# Autodesk Inventor assembly: 2803622 EAMM-U-145-D100-120G-188-S1
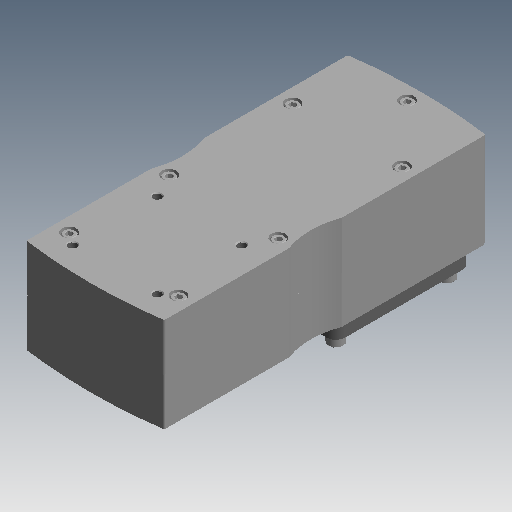
[picture p0: Inventor's stored thumbnail of the model, 512x512]
Saved by Autodesk Inventor 2021 (Build 250183000, 183)
## iProperties
Category: PARTsolutions
Company: FESTO
Part Number: 2803622 EAMM-U-145-D100-120G-188-S1
Catalog Web Link: www.cadenas.de
Description: EAMM-U-parallel kit
Vendor: FESTO
Document SubType Name: Assembly
Designer: partserver
Manufacturer: FESTO
Mass: 12100 g
Surface Area: 4483.28 cm^2
Volume: 3170.64 cm^3
Density: 3.81626 g/cm^3
PSOL_IDENT_0: {ATYP=ASSISTANT},{DATA=script=$CADENAS_DATA/23d-libs/festo/webfesto.vbb&M_FAMILY=EAMM&M_GROUP=01&M_P
PSOL_IDENT_1: ARTNO=2803622&IDCODE1=EAMM-U-145-D100-120G-188-S1&IDCODE2=&customer_number_cns=&MATES=1&LOD=HI&LOCKE
PSOL_IDENT_2: RP=0&SINGLEPART=1}
NB: 2803622 EAMM-U-145-D100-120G-188-S1
NN: EAMM-U
NT: parallel kit
NBSYN: $TNR. $TYP.
LINA: 2803622 EAMM-U-145-D100-120G-188-S1
CATALOG: Festo
TNR: 2803622
TYP: EAMM-U-145-D100-120G-188-S1
B1: 145
B2: 0
B3: 89
B4: 0
B5: 89
B6: 115
D1: 80
D2: 100
D3: 100
D4: 11
D5: 11
D6: M10
D7: 0
H1: 348
H2: 0
H3: 89
H4: 0
H5: 89
H6: 70
H7: 188
H8: 35
H9: 70
H10: 193
H11: 130
H12: 5
L1: 99.5
L2: 0.5
L3: 0
L4: 0
T1: 25
W1: 45
W2: 0
CNSMASSEXACT: 12.1
SUPPLIER: FESTO
ARTICLENO: 2803622 EAMM-U-145-D100-120G-188-S1
BOMINFO: 2803622 EAMM-U-145-D100-120G-188-S1
CREATOR: CADENAS GmbH
Title: 2803622 EAMM-U-145-D100-120G-188-S1
Author: Cadenas PARTsolutions
Comments: parallel kit
## Documents named in this file (11)
- C:\Users\Santiago Suárez\Documents\GitHub\Dis.-Mecatronico-E6\inventor proyecto\PARTserver0202108060004321756159710e898ce\AIS2021\2803622 EAMM-U-145-D100-120G-188-S1.iam
- C:\Users\Santiago Suárez\Documents\GitHub\Dis.-Mecatronico-E6\inventor proyecto\PARTserver0202108060004321756159710e898ce\AIS2021\1465008 EAMM-U-145-D100-140A-348S---(UT).ipt
- C:\Users\Santiago Suárez\Documents\GitHub\Dis.-Mecatronico-E6\inventor proyecto\PARTserver0202108060004321756159710e898ce\AIS2021\1464690 EAMM-U-145-D100-___-348S---(OT).ipt
- C:\Users\Santiago Suárez\Documents\GitHub\Dis.-Mecatronico-E6\inventor proyecto\PARTserver0202108060004321756159710e898ce\AIS2021\DIN-912 - M8x50(F).ipt
- C:\Users\Santiago Suárez\Documents\GitHub\Dis.-Mecatronico-E6\inventor proyecto\PARTserver0202108060004321756159710e898ce\AIS2021\DIN 557 - M10.ipt
- C:\Users\Santiago Suárez\Documents\GitHub\Dis.-Mecatronico-E6\inventor proyecto\PARTserver0202108060004321756159710e898ce\AIS2021\1451339 M10-NBR-10x16_9x1_5.ipt
- C:\Users\Santiago Suárez\Documents\GitHub\Dis.-Mecatronico-E6\inventor proyecto\PARTserver0202108060004321756159710e898ce\AIS2021\DIN-6912 - M10x20(F).ipt
- C:\Users\Santiago Suárez\Documents\GitHub\Dis.-Mecatronico-E6\inventor proyecto\PARTserver0202108060004321756159710e898ce\AIS2021\2683767 EAMF-U-140A-120G-S1---(ADAX).ipt
- C:\Users\Santiago Suárez\Documents\GitHub\Dis.-Mecatronico-E6\inventor proyecto\PARTserver0202108060004321756159710e898ce\AIS2021\DIN-912 - M10x20(F).ipt
- C:\Users\Santiago Suárez\Documents\GitHub\Dis.-Mecatronico-E6\inventor proyecto\PARTserver0202108060004321756159710e898ce\AIS2021\DIN-912 - M10x55(F).ipt
- C:\Users\Santiago Suárez\Documents\GitHub\Dis.-Mecatronico-E6\inventor proyecto\PARTserver0202108060004321756159710e898ce\AIS2021\706368 GPN.ipt
## Components (35 placed, 10 different names)
1. 1465008 EAMM-U-145-D100-140A-348S---(UT):1 — AS_1_XY@1 <-> ANBAU2_XY@14, AS_1_Z@1 <-> ANBAU2_Z@14, AS_1_YZ@1 <-> ANBAU2_YZ@14, AS_2_XY@1 <-> ANBAU2_XY@15, AS_2_Z@1 <-> ANBAU2_Z@15, AS_2_YZ@1 <-> ANBAU2_YZ@15, AS_3_XY@1 <-> ANBAU2_XY@16, AS_3_Z@1 <-> ANBAU2_Z@16, AS_3_YZ@1 <-> ANBAU2_YZ@16, AS_4_XY@1 <-> ANBAU2_XY@17, AS_4_Z@1 <-> ANBAU2_Z@17, AS_4_YZ@1 <-> ANBAU2_YZ@17, AS_1_XY@1 <-> MONTAGE_XY@18, AS_1_Z@1 <-> MONTAGE_Z@18, AS_1_YZ@1 <-> MONTAGE_YZ@18, AS_2_XY@1 <-> MONTAGE_XY@19, AS_2_Z@1 <-> MONTAGE_Z@19, AS_2_YZ@1 <-> MONTAGE_YZ@19, AS_3_XY@1 <-> MONTAGE_XY@20, AS_3_Z@1 <-> MONTAGE_Z@20, AS_3_YZ@1 <-> MONTAGE_YZ@20, AS_4_XY@1 <-> MONTAGE_XY@21, AS_4_Z@1 <-> MONTAGE_Z@21, AS_4_YZ@1 <-> MONTAGE_YZ@21, DM_XY@1 <-> ANBAU_XY@22, DM_Z@1 <-> ANBAU_Z@22, DM_YZ@1 <-> ANBAU_YZ@22, MS_1_XY@1 <-> ANBAU_XY@27, MS_1_Z@1 <-> ANBAU_Z@27, MS_1_YZ@1 <-> ANBAU_YZ@27, MS_2_XY@1 <-> ANBAU_XY@28, MS_2_Z@1 <-> ANBAU_Z@28, MS_2_YZ@1 <-> ANBAU_YZ@28, MS_3_XY@1 <-> ANBAU_XY@29, MS_3_Z@1 <-> ANBAU_Z@29, MS_3_YZ@1 <-> ANBAU_YZ@29, MS_4_XY@1 <-> ANBAU_XY@30, MS_4_Z@1 <-> ANBAU_Z@30, MS_4_YZ@1 <-> ANBAU_YZ@30, MS_1_XY@1 <-> ANBAU1_XY@31, MS_1_Z@1 <-> ANBAU1_Z@31, MS_1_YZ@1 <-> ANBAU1_YZ@31, MS_2_XY@1 <-> ANBAU1_XY@32, MS_2_Z@1 <-> ANBAU1_Z@32, MS_2_YZ@1 <-> ANBAU1_YZ@32, MS_3_XY@1 <-> ANBAU1_XY@33, MS_3_Z@1 <-> ANBAU1_Z@33, MS_3_YZ@1 <-> ANBAU1_YZ@33, MS_4_XY@1 <-> ANBAU1_XY@34, MS_4_Z@1 <-> ANBAU1_Z@34, MS_4_YZ@1 <-> ANBAU1_YZ@34, VS_XY@1 <-> ANBAU_XY@35, VS_Z@1 <-> ANBAU_Z@35, VS_YZ@1 <-> ANBAU_YZ@35
2. 1464690 EAMM-U-145-D100-___-348S---(OT):1
3. DIN-912 - M8x50(F):1
4. DIN-912 - M8x50(F):2
5. DIN-912 - M8x50(F):3
6. DIN-912 - M8x50(F):4
7. DIN-912 - M8x50(F):5
8. DIN-912 - M8x50(F):6
9. DIN-912 - M8x50(F):7
10. DIN 557 - M10:1
11. DIN 557 - M10:2
12. DIN 557 - M10:3
13. DIN 557 - M10:4
14. 1451339 M10-NBR-10x16_9x1_5:1 — AS_1_XY@1 <-> ANBAU2_XY@14, AS_1_Z@1 <-> ANBAU2_Z@14, AS_1_YZ@1 <-> ANBAU2_YZ@14
15. 1451339 M10-NBR-10x16_9x1_5:2 — AS_2_XY@1 <-> ANBAU2_XY@15, AS_2_Z@1 <-> ANBAU2_Z@15, AS_2_YZ@1 <-> ANBAU2_YZ@15
16. 1451339 M10-NBR-10x16_9x1_5:3 — AS_3_XY@1 <-> ANBAU2_XY@16, AS_3_Z@1 <-> ANBAU2_Z@16, AS_3_YZ@1 <-> ANBAU2_YZ@16
17. 1451339 M10-NBR-10x16_9x1_5:4 — AS_4_XY@1 <-> ANBAU2_XY@17, AS_4_Z@1 <-> ANBAU2_Z@17, AS_4_YZ@1 <-> ANBAU2_YZ@17
18. DIN-6912 - M10x20(F):1 — AS_1_XY@1 <-> MONTAGE_XY@18, AS_1_Z@1 <-> MONTAGE_Z@18, AS_1_YZ@1 <-> MONTAGE_YZ@18
19. DIN-6912 - M10x20(F):2 — AS_2_XY@1 <-> MONTAGE_XY@19, AS_2_Z@1 <-> MONTAGE_Z@19, AS_2_YZ@1 <-> MONTAGE_YZ@19
20. DIN-6912 - M10x20(F):3 — AS_3_XY@1 <-> MONTAGE_XY@20, AS_3_Z@1 <-> MONTAGE_Z@20, AS_3_YZ@1 <-> MONTAGE_YZ@20
21. DIN-6912 - M10x20(F):4 — AS_4_XY@1 <-> MONTAGE_XY@21, AS_4_Z@1 <-> MONTAGE_Z@21, AS_4_YZ@1 <-> MONTAGE_YZ@21
22. 2683767 EAMF-U-140A-120G-S1---(ADAX):1 — DM_XY@1 <-> ANBAU_XY@22, DM_Z@1 <-> ANBAU_Z@22, DM_YZ@1 <-> ANBAU_YZ@22, M_SCREWS_1_XY@22 <-> ANBAU_XY@23, M_SCREWS_1_Z@22 <-> ANBAU_Z@23, M_SCREWS_1_YZ@22 <-> ANBAU_YZ@23, M_SCREWS_2_XY@22 <-> ANBAU_XY@24, M_SCREWS_2_Z@22 <-> ANBAU_Z@24, M_SCREWS_2_YZ@22 <-> ANBAU_YZ@24, M_SCREWS_3_XY@22 <-> ANBAU_XY@25, M_SCREWS_3_Z@22 <-> ANBAU_Z@25, M_SCREWS_3_YZ@22 <-> ANBAU_YZ@25, M_SCREWS_4_XY@22 <-> ANBAU_XY@26, M_SCREWS_4_Z@22 <-> ANBAU_Z@26, M_SCREWS_4_YZ@22 <-> ANBAU_YZ@26
23. DIN-912 - M10x20(F):1 — M_SCREWS_1_XY@22 <-> ANBAU_XY@23, M_SCREWS_1_Z@22 <-> ANBAU_Z@23, M_SCREWS_1_YZ@22 <-> ANBAU_YZ@23
24. DIN-912 - M10x20(F):2 — M_SCREWS_2_XY@22 <-> ANBAU_XY@24, M_SCREWS_2_Z@22 <-> ANBAU_Z@24, M_SCREWS_2_YZ@22 <-> ANBAU_YZ@24
25. DIN-912 - M10x20(F):3 — M_SCREWS_3_XY@22 <-> ANBAU_XY@25, M_SCREWS_3_Z@22 <-> ANBAU_Z@25, M_SCREWS_3_YZ@22 <-> ANBAU_YZ@25
26. DIN-912 - M10x20(F):4 — M_SCREWS_4_XY@22 <-> ANBAU_XY@26, M_SCREWS_4_Z@22 <-> ANBAU_Z@26, M_SCREWS_4_YZ@22 <-> ANBAU_YZ@26
27. DIN-912 - M10x55(F):1 — MS_1_XY@1 <-> ANBAU_XY@27, MS_1_Z@1 <-> ANBAU_Z@27, MS_1_YZ@1 <-> ANBAU_YZ@27
28. DIN-912 - M10x55(F):2 — MS_2_XY@1 <-> ANBAU_XY@28, MS_2_Z@1 <-> ANBAU_Z@28, MS_2_YZ@1 <-> ANBAU_YZ@28
29. DIN-912 - M10x55(F):3 — MS_3_XY@1 <-> ANBAU_XY@29, MS_3_Z@1 <-> ANBAU_Z@29, MS_3_YZ@1 <-> ANBAU_YZ@29
30. DIN-912 - M10x55(F):4 — MS_4_XY@1 <-> ANBAU_XY@30, MS_4_Z@1 <-> ANBAU_Z@30, MS_4_YZ@1 <-> ANBAU_YZ@30
31. 1451339 M10-NBR-10x16_9x1_5:5 — MS_1_XY@1 <-> ANBAU1_XY@31, MS_1_Z@1 <-> ANBAU1_Z@31, MS_1_YZ@1 <-> ANBAU1_YZ@31
32. 1451339 M10-NBR-10x16_9x1_5:6 — MS_2_XY@1 <-> ANBAU1_XY@32, MS_2_Z@1 <-> ANBAU1_Z@32, MS_2_YZ@1 <-> ANBAU1_YZ@32
33. 1451339 M10-NBR-10x16_9x1_5:7 — MS_3_XY@1 <-> ANBAU1_XY@33, MS_3_Z@1 <-> ANBAU1_Z@33, MS_3_YZ@1 <-> ANBAU1_YZ@33
34. 1451339 M10-NBR-10x16_9x1_5:8 — MS_4_XY@1 <-> ANBAU1_XY@34, MS_4_Z@1 <-> ANBAU1_Z@34, MS_4_YZ@1 <-> ANBAU1_YZ@34
35. 706368 GPN:1 — VS_XY@1 <-> ANBAU_XY@35, VS_Z@1 <-> ANBAU_Z@35, VS_YZ@1 <-> ANBAU_YZ@35
## Relationships (66: Mate 44, Angle 22)
- AS_1_XY@1 <-> ANBAU2_XY@14 [Mate]: 1465008 EAMM-U-145-D100-140A-348S---(UT):1 ↔ 1451339 M10-NBR-10x16_9x1_5:1
- AS_1_Z@1 <-> ANBAU2_Z@14 [Mate]: 1465008 EAMM-U-145-D100-140A-348S---(UT):1 ↔ 1451339 M10-NBR-10x16_9x1_5:1
- AS_1_YZ@1 <-> ANBAU2_YZ@14 [Angle] (0 deg): 1465008 EAMM-U-145-D100-140A-348S---(UT):1 ↔ 1451339 M10-NBR-10x16_9x1_5:1
- AS_2_XY@1 <-> ANBAU2_XY@15 [Mate]: 1465008 EAMM-U-145-D100-140A-348S---(UT):1 ↔ 1451339 M10-NBR-10x16_9x1_5:2
- AS_2_Z@1 <-> ANBAU2_Z@15 [Mate]: 1465008 EAMM-U-145-D100-140A-348S---(UT):1 ↔ 1451339 M10-NBR-10x16_9x1_5:2
- AS_2_YZ@1 <-> ANBAU2_YZ@15 [Angle] (0 deg): 1465008 EAMM-U-145-D100-140A-348S---(UT):1 ↔ 1451339 M10-NBR-10x16_9x1_5:2
- AS_3_XY@1 <-> ANBAU2_XY@16 [Mate]: 1465008 EAMM-U-145-D100-140A-348S---(UT):1 ↔ 1451339 M10-NBR-10x16_9x1_5:3
- AS_3_Z@1 <-> ANBAU2_Z@16 [Mate]: 1465008 EAMM-U-145-D100-140A-348S---(UT):1 ↔ 1451339 M10-NBR-10x16_9x1_5:3
- AS_3_YZ@1 <-> ANBAU2_YZ@16 [Angle] (0 deg): 1465008 EAMM-U-145-D100-140A-348S---(UT):1 ↔ 1451339 M10-NBR-10x16_9x1_5:3
- AS_4_XY@1 <-> ANBAU2_XY@17 [Mate]: 1465008 EAMM-U-145-D100-140A-348S---(UT):1 ↔ 1451339 M10-NBR-10x16_9x1_5:4
- AS_4_Z@1 <-> ANBAU2_Z@17 [Mate]: 1465008 EAMM-U-145-D100-140A-348S---(UT):1 ↔ 1451339 M10-NBR-10x16_9x1_5:4
- AS_4_YZ@1 <-> ANBAU2_YZ@17 [Angle] (0 deg): 1465008 EAMM-U-145-D100-140A-348S---(UT):1 ↔ 1451339 M10-NBR-10x16_9x1_5:4
- AS_1_XY@1 <-> MONTAGE_XY@18 [Mate] (2.5 mm): 1465008 EAMM-U-145-D100-140A-348S---(UT):1 ↔ DIN-6912 - M10x20(F):1
- AS_1_Z@1 <-> MONTAGE_Z@18 [Mate]: 1465008 EAMM-U-145-D100-140A-348S---(UT):1 ↔ DIN-6912 - M10x20(F):1
- AS_1_YZ@1 <-> MONTAGE_YZ@18 [Angle] (0 deg): 1465008 EAMM-U-145-D100-140A-348S---(UT):1 ↔ DIN-6912 - M10x20(F):1
- AS_2_XY@1 <-> MONTAGE_XY@19 [Mate] (2.5 mm): 1465008 EAMM-U-145-D100-140A-348S---(UT):1 ↔ DIN-6912 - M10x20(F):2
- AS_2_Z@1 <-> MONTAGE_Z@19 [Mate]: 1465008 EAMM-U-145-D100-140A-348S---(UT):1 ↔ DIN-6912 - M10x20(F):2
- AS_2_YZ@1 <-> MONTAGE_YZ@19 [Angle] (0 deg): 1465008 EAMM-U-145-D100-140A-348S---(UT):1 ↔ DIN-6912 - M10x20(F):2
- AS_3_XY@1 <-> MONTAGE_XY@20 [Mate] (2.5 mm): 1465008 EAMM-U-145-D100-140A-348S---(UT):1 ↔ DIN-6912 - M10x20(F):3
- AS_3_Z@1 <-> MONTAGE_Z@20 [Mate]: 1465008 EAMM-U-145-D100-140A-348S---(UT):1 ↔ DIN-6912 - M10x20(F):3
- AS_3_YZ@1 <-> MONTAGE_YZ@20 [Angle] (0 deg): 1465008 EAMM-U-145-D100-140A-348S---(UT):1 ↔ DIN-6912 - M10x20(F):3
- AS_4_XY@1 <-> MONTAGE_XY@21 [Mate] (2.5 mm): 1465008 EAMM-U-145-D100-140A-348S---(UT):1 ↔ DIN-6912 - M10x20(F):4
- AS_4_Z@1 <-> MONTAGE_Z@21 [Mate]: 1465008 EAMM-U-145-D100-140A-348S---(UT):1 ↔ DIN-6912 - M10x20(F):4
- AS_4_YZ@1 <-> MONTAGE_YZ@21 [Angle] (0 deg): 1465008 EAMM-U-145-D100-140A-348S---(UT):1 ↔ DIN-6912 - M10x20(F):4
- DM_XY@1 <-> ANBAU_XY@22 [Mate] (-0.5 mm): 1465008 EAMM-U-145-D100-140A-348S---(UT):1 ↔ 2683767 EAMF-U-140A-120G-S1---(ADAX):1
- DM_Z@1 <-> ANBAU_Z@22 [Mate]: 1465008 EAMM-U-145-D100-140A-348S---(UT):1 ↔ 2683767 EAMF-U-140A-120G-S1---(ADAX):1
- DM_YZ@1 <-> ANBAU_YZ@22 [Angle] (0 deg): 1465008 EAMM-U-145-D100-140A-348S---(UT):1 ↔ 2683767 EAMF-U-140A-120G-S1---(ADAX):1
- M_SCREWS_1_XY@22 <-> ANBAU_XY@23 [Mate]: 2683767 EAMF-U-140A-120G-S1---(ADAX):1 ↔ DIN-912 - M10x20(F):1
- M_SCREWS_1_Z@22 <-> ANBAU_Z@23 [Mate]: 2683767 EAMF-U-140A-120G-S1---(ADAX):1 ↔ DIN-912 - M10x20(F):1
- M_SCREWS_1_YZ@22 <-> ANBAU_YZ@23 [Angle] (0 deg): 2683767 EAMF-U-140A-120G-S1---(ADAX):1 ↔ DIN-912 - M10x20(F):1
- M_SCREWS_2_XY@22 <-> ANBAU_XY@24 [Mate]: 2683767 EAMF-U-140A-120G-S1---(ADAX):1 ↔ DIN-912 - M10x20(F):2
- M_SCREWS_2_Z@22 <-> ANBAU_Z@24 [Mate]: 2683767 EAMF-U-140A-120G-S1---(ADAX):1 ↔ DIN-912 - M10x20(F):2
- M_SCREWS_2_YZ@22 <-> ANBAU_YZ@24 [Angle] (0 deg): 2683767 EAMF-U-140A-120G-S1---(ADAX):1 ↔ DIN-912 - M10x20(F):2
- M_SCREWS_3_XY@22 <-> ANBAU_XY@25 [Mate]: 2683767 EAMF-U-140A-120G-S1---(ADAX):1 ↔ DIN-912 - M10x20(F):3
- M_SCREWS_3_Z@22 <-> ANBAU_Z@25 [Mate]: 2683767 EAMF-U-140A-120G-S1---(ADAX):1 ↔ DIN-912 - M10x20(F):3
- M_SCREWS_3_YZ@22 <-> ANBAU_YZ@25 [Angle] (0 deg): 2683767 EAMF-U-140A-120G-S1---(ADAX):1 ↔ DIN-912 - M10x20(F):3
- M_SCREWS_4_XY@22 <-> ANBAU_XY@26 [Mate]: 2683767 EAMF-U-140A-120G-S1---(ADAX):1 ↔ DIN-912 - M10x20(F):4
- M_SCREWS_4_Z@22 <-> ANBAU_Z@26 [Mate]: 2683767 EAMF-U-140A-120G-S1---(ADAX):1 ↔ DIN-912 - M10x20(F):4
- M_SCREWS_4_YZ@22 <-> ANBAU_YZ@26 [Angle] (0 deg): 2683767 EAMF-U-140A-120G-S1---(ADAX):1 ↔ DIN-912 - M10x20(F):4
- MS_1_XY@1 <-> ANBAU_XY@27 [Mate] (-2.5 mm): 1465008 EAMM-U-145-D100-140A-348S---(UT):1 ↔ DIN-912 - M10x55(F):1
- MS_1_Z@1 <-> ANBAU_Z@27 [Mate]: 1465008 EAMM-U-145-D100-140A-348S---(UT):1 ↔ DIN-912 - M10x55(F):1
- MS_1_YZ@1 <-> ANBAU_YZ@27 [Angle] (0 deg): 1465008 EAMM-U-145-D100-140A-348S---(UT):1 ↔ DIN-912 - M10x55(F):1
- MS_2_XY@1 <-> ANBAU_XY@28 [Mate] (-2.5 mm): 1465008 EAMM-U-145-D100-140A-348S---(UT):1 ↔ DIN-912 - M10x55(F):2
- MS_2_Z@1 <-> ANBAU_Z@28 [Mate]: 1465008 EAMM-U-145-D100-140A-348S---(UT):1 ↔ DIN-912 - M10x55(F):2
- MS_2_YZ@1 <-> ANBAU_YZ@28 [Angle] (0 deg): 1465008 EAMM-U-145-D100-140A-348S---(UT):1 ↔ DIN-912 - M10x55(F):2
- MS_3_XY@1 <-> ANBAU_XY@29 [Mate] (-2.5 mm): 1465008 EAMM-U-145-D100-140A-348S---(UT):1 ↔ DIN-912 - M10x55(F):3
- MS_3_Z@1 <-> ANBAU_Z@29 [Mate]: 1465008 EAMM-U-145-D100-140A-348S---(UT):1 ↔ DIN-912 - M10x55(F):3
- MS_3_YZ@1 <-> ANBAU_YZ@29 [Angle] (0 deg): 1465008 EAMM-U-145-D100-140A-348S---(UT):1 ↔ DIN-912 - M10x55(F):3
- MS_4_XY@1 <-> ANBAU_XY@30 [Mate] (-2.5 mm): 1465008 EAMM-U-145-D100-140A-348S---(UT):1 ↔ DIN-912 - M10x55(F):4
- MS_4_Z@1 <-> ANBAU_Z@30 [Mate]: 1465008 EAMM-U-145-D100-140A-348S---(UT):1 ↔ DIN-912 - M10x55(F):4
- MS_4_YZ@1 <-> ANBAU_YZ@30 [Angle] (0 deg): 1465008 EAMM-U-145-D100-140A-348S---(UT):1 ↔ DIN-912 - M10x55(F):4
- MS_1_XY@1 <-> ANBAU1_XY@31 [Mate]: 1465008 EAMM-U-145-D100-140A-348S---(UT):1 ↔ 1451339 M10-NBR-10x16_9x1_5:5
- MS_1_Z@1 <-> ANBAU1_Z@31 [Mate]: 1465008 EAMM-U-145-D100-140A-348S---(UT):1 ↔ 1451339 M10-NBR-10x16_9x1_5:5
- MS_1_YZ@1 <-> ANBAU1_YZ@31 [Angle] (0 deg): 1465008 EAMM-U-145-D100-140A-348S---(UT):1 ↔ 1451339 M10-NBR-10x16_9x1_5:5
- MS_2_XY@1 <-> ANBAU1_XY@32 [Mate]: 1465008 EAMM-U-145-D100-140A-348S---(UT):1 ↔ 1451339 M10-NBR-10x16_9x1_5:6
- MS_2_Z@1 <-> ANBAU1_Z@32 [Mate]: 1465008 EAMM-U-145-D100-140A-348S---(UT):1 ↔ 1451339 M10-NBR-10x16_9x1_5:6
- MS_2_YZ@1 <-> ANBAU1_YZ@32 [Angle] (0 deg): 1465008 EAMM-U-145-D100-140A-348S---(UT):1 ↔ 1451339 M10-NBR-10x16_9x1_5:6
- MS_3_XY@1 <-> ANBAU1_XY@33 [Mate]: 1465008 EAMM-U-145-D100-140A-348S---(UT):1 ↔ 1451339 M10-NBR-10x16_9x1_5:7
- MS_3_Z@1 <-> ANBAU1_Z@33 [Mate]: 1465008 EAMM-U-145-D100-140A-348S---(UT):1 ↔ 1451339 M10-NBR-10x16_9x1_5:7
- MS_3_YZ@1 <-> ANBAU1_YZ@33 [Angle] (0 deg): 1465008 EAMM-U-145-D100-140A-348S---(UT):1 ↔ 1451339 M10-NBR-10x16_9x1_5:7
- MS_4_XY@1 <-> ANBAU1_XY@34 [Mate]: 1465008 EAMM-U-145-D100-140A-348S---(UT):1 ↔ 1451339 M10-NBR-10x16_9x1_5:8
- MS_4_Z@1 <-> ANBAU1_Z@34 [Mate]: 1465008 EAMM-U-145-D100-140A-348S---(UT):1 ↔ 1451339 M10-NBR-10x16_9x1_5:8
- MS_4_YZ@1 <-> ANBAU1_YZ@34 [Angle] (0 deg): 1465008 EAMM-U-145-D100-140A-348S---(UT):1 ↔ 1451339 M10-NBR-10x16_9x1_5:8
- VS_XY@1 <-> ANBAU_XY@35 [Mate]: 1465008 EAMM-U-145-D100-140A-348S---(UT):1 ↔ 706368 GPN:1
- VS_Z@1 <-> ANBAU_Z@35 [Mate]: 1465008 EAMM-U-145-D100-140A-348S---(UT):1 ↔ 706368 GPN:1
- VS_YZ@1 <-> ANBAU_YZ@35 [Angle] (0 deg): 1465008 EAMM-U-145-D100-140A-348S---(UT):1 ↔ 706368 GPN:1
